# Autodesk Inventor assembly: mill_assembly
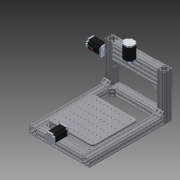
[picture p0: Inventor's stored thumbnail of the model, 180x180]
Saved by Autodesk Inventor 2014 (Build 180170000, 170)
## iProperties
Created: 2014-08-08
Part Number: mill_assembly
Document SubType Name: Assembly
Designer: Matthew
Author: Matthew
## Documents named in this file (9)
- C:\Users\Matthew\Documents\GitHub\CNC Mill\mill_assembly.iam
- C:\Users\Matthew\Documents\GitHub\CNC Mill\Imported Components\8020-2040\Assembly2.iam
- C:\Users\Matthew\Documents\GitHub\CNC Mill\2020.ipt
- C:\Users\Matthew\Documents\GitHub\CNC Mill\2020_18in.ipt
- C:\Users\Matthew\Documents\GitHub\CNC Mill\plate_4127.ipt
- C:\Users\Matthew\Documents\GitHub\CNC Mill\gusset_4138.ipt
- C:\Users\Matthew\Documents\GitHub\CNC Mill\gusset_4134.ipt
- C:\Users\Matthew\Documents\GitHub\CNC Mill\Imported Components\425oz stepper motor\425oz stepper motor.ipt
- C:\Users\Matthew\Documents\GitHub\CNC Mill\mic6_plate.ipt
## Components (21 placed, 8 different names)
1. Assembly2:1 [sub-assembly] — Mate:13, Flush:1, Flush:2, Mate:16, Flush:4, Flush:5, Mate:22, Mate:24, Mate:26, Mate:39, Mate:41, Mate:42, Mate:43, Mate:45, Mate:52
2. 2020:1 — Mate:13, Flush:1, Flush:2, Mate:17, Flush:6, Flush:7, Mate:25, Mate:30, Mate:44
3. 2020:2 — Mate:16, Flush:4, Flush:5, Mate:18, Flush:8, Flush:9, Mate:19, Flush:10, Flush:11, Mate:21, Mate:23, Mate:27, Mate:40, Mate:53
4. 2020_18in:1 — Mate:17, Flush:6, Flush:7, Mate:31, Mate:32, Mate:38, Mate:47, Mate:48
5. 2020_18in:2 — Mate:18, Flush:8, Flush:9, Flush:12, Mate:20, Flush:13, Mate:28, Mate:29, Mate:34, Mate:50, Mate:51, Mate:54
6. 2020:3 — Mate:19, Flush:10, Flush:11, Mate:46, Mate:49
7. 2020:4 — Flush:12, Mate:20, Flush:13, Mate:33, Mate:35, Mate:36, Mate:37, Flush:14
8. plate_4127:1 — Mate:39, Mate:40, Mate:41
9. gusset_4138:1 — Mate:21, Mate:22, Mate:23
10. gusset_4134:1 — Mate:27, Mate:28, Mate:29
11. gusset_4138:2 — Mate:24, Mate:25, Mate:26
12. gusset_4134:2 — Mate:30, Mate:31, Mate:32
13. gusset_4134:3 — Mate:33, Mate:34, Mate:35
14. gusset_4134:4 — Mate:36, Mate:37, Mate:38
15. plate_4127:2 — Mate:42, Mate:43, Mate:44, Mate:45
16. gusset_4134:5 — Mate:49, Mate:50, Mate:51
17. gusset_4134:6 — Mate:46, Mate:47, Mate:48
18. 425oz stepper motor:1 — Mate:52
19. 425oz stepper motor:2 — Flush:14
20. 425oz stepper motor:3 — Mate:53
21. mic6_plate:1 — Mate:54
## Relationships (53: Mate 40, Flush 13)
- Mate:13: Assembly2:1 ↔ 2020:1
- Flush:1: Assembly2:1 ↔ 2020:1
- Flush:2: Assembly2:1 ↔ 2020:1
- Mate:16: Assembly2:1 ↔ 2020:2
- Flush:4: Assembly2:1 ↔ 2020:2
- Flush:5: Assembly2:1 ↔ 2020:2
- Mate:17: 2020:1 ↔ 2020_18in:1
- Flush:6: 2020:1 ↔ 2020_18in:1
- Flush:7: 2020:1 ↔ 2020_18in:1
- Mate:18: 2020:2 ↔ 2020_18in:2
- Flush:8: 2020:2 ↔ 2020_18in:2
- Flush:9: 2020:2 ↔ 2020_18in:2
- Mate:19: 2020:2 ↔ 2020:3
- Flush:10: 2020:2 ↔ 2020:3
- Flush:11: 2020:2 ↔ 2020:3
- Flush:12: 2020_18in:2 ↔ 2020:4
- Mate:20: 2020_18in:2 ↔ 2020:4
- Flush:13: 2020_18in:2 ↔ 2020:4
- Mate:21: 2020:2 ↔ gusset_4138:1
- Mate:22: Assembly2:1 ↔ gusset_4138:1
- Mate:23: 2020:2 ↔ gusset_4138:1
- Mate:24: Assembly2:1 ↔ gusset_4138:2
- Mate:25: 2020:1 ↔ gusset_4138:2
- Mate:26: Assembly2:1 ↔ gusset_4138:2
- Mate:27: 2020:2 ↔ gusset_4134:1
- Mate:28: 2020_18in:2 ↔ gusset_4134:1
- Mate:29: 2020_18in:2 ↔ gusset_4134:1
- Mate:30: 2020:1 ↔ gusset_4134:2
- Mate:31: 2020_18in:1 ↔ gusset_4134:2
- Mate:32: 2020_18in:1 ↔ gusset_4134:2
- Mate:33: 2020:4 ↔ gusset_4134:3
- Mate:34: 2020_18in:2 ↔ gusset_4134:3
- Mate:35: 2020:4 ↔ gusset_4134:3
- Mate:36: 2020:4 ↔ gusset_4134:4
- Mate:37: 2020:4 ↔ gusset_4134:4
- Mate:38: 2020_18in:1 ↔ gusset_4134:4
- Mate:39: Assembly2:1 ↔ plate_4127:1
- Mate:40: 2020:2 ↔ plate_4127:1
- Mate:41: Assembly2:1 ↔ plate_4127:1
- Mate:42: Assembly2:1 ↔ plate_4127:2
- Mate:43: Assembly2:1 ↔ plate_4127:2
- Mate:44: 2020:1 ↔ plate_4127:2
- Mate:45: Assembly2:1 ↔ plate_4127:2
- Mate:46: 2020:3 ↔ gusset_4134:6
- Mate:47: 2020_18in:1 ↔ gusset_4134:6
- Mate:48: 2020_18in:1 ↔ gusset_4134:6
- Mate:49: 2020:3 ↔ gusset_4134:5
- Mate:50: 2020_18in:2 ↔ gusset_4134:5
- Mate:51: 2020_18in:2 ↔ gusset_4134:5
- Mate:52: Assembly2:1 ↔ 425oz stepper motor:1
- Mate:53: 2020:2 ↔ 425oz stepper motor:3
- Flush:14: 2020:4 ↔ 425oz stepper motor:2
- Mate:54: 2020_18in:2 ↔ mic6_plate:1
